# Autodesk Inventor assembly: CARCASA_ESTRUCTURA_Y_CHAPAS
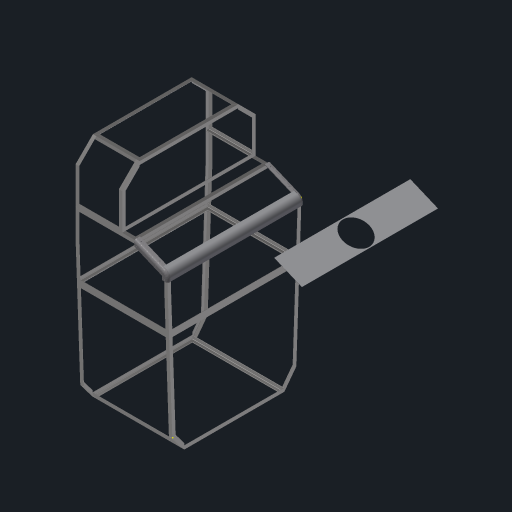
[picture p0: Inventor's stored thumbnail of the model, 512x512]
Saved by Autodesk Inventor 2024.3 (Build 283343000, 343)
## iProperties
Created: 2024-05-18
Part Number: CARCASA_ESTRUCTURA_Y_CHAPAS
Material: Generic
Document SubType Name: Assembly
Designer: Niler
Author: Niler
## Documents named in this file (11)
- C:\Users\Niler\OneDrive\Escritorio\RECICLADOR\RECICLADOR_MODELO_3D\VERSION_3_COMPLETA\CARCASA_ESTRUCTURA_Y_CHAPAS.iam
- C:\Users\Niler\OneDrive\Escritorio\RECICLADOR\RECICLADOR_MODELO_3D\VERSION_3_COMPLETA\ESTRUCTURA\ESTRUCTURA_COMPLETA.iam
- C:\Users\Niler\OneDrive\Escritorio\RECICLADOR\RECICLADOR_MODELO_3D\VERSION_3_COMPLETA\PIEZAS_CHAPAS_ALUMINIO\CARCASA_ALUM_2.ipt
- C:\Users\Niler\OneDrive\Escritorio\RECICLADOR\RECICLADOR_MODELO_3D\VERSION_3_COMPLETA\ESQUINAS\ESQUINA_REDONDEADA_R20_P1.ipt
- C:\Users\Niler\OneDrive\Escritorio\RECICLADOR\RECICLADOR_MODELO_3D\VERSION_3_COMPLETA\ESQUINAS\ESQUINA_REDONDEADA_R20_P2.ipt
- C:\Users\Niler\OneDrive\Escritorio\RECICLADOR\RECICLADOR_MODELO_3D\VERSION_3_COMPLETA\ESQUINAS\ESQUINA_REDONDEADA_R20_P3.ipt
- C:\Users\Niler\OneDrive\Escritorio\RECICLADOR\RECICLADOR_MODELO_3D\ESQUINA_REDONDEADA_R50.ipt
- C:\Users\Niler\OneDrive\Escritorio\RECICLADOR\RECICLADOR_MODELO_3D\ESQUINA_REDONDEADA_R50_P2.ipt
- C:\Users\Niler\OneDrive\Escritorio\RECICLADOR\RECICLADOR_MODELO_3D\VERSION_3_COMPLETA\ESQUINAS\ESQUINA_REDONDEADA_R20_P1_MIR.ipt
- C:\Users\Niler\OneDrive\Escritorio\RECICLADOR\RECICLADOR_MODELO_3D\VERSION_3_COMPLETA\ESQUINAS\ESQUINA_REDONDEADA_R20_P2_MIR.ipt
- C:\Users\Niler\OneDrive\Escritorio\RECICLADOR\RECICLADOR_MODELO_3D\VERSION_3_COMPLETA\ESQUINAS\ESQUINA_REDONDEADA_R20_P3_MIR.ipt
## Components (16 placed, 10 different names)
1. ESTRUCTURA_COMPLETA:1 [sub-assembly] — Mate:1, Mate:2, Angle:1, Mate:3, Angle:2, Mate:9, Mate:10, Mate:11, Mate:16, Mate:17, Mate:22, Mate:23, Mate:24, Mate:25
2. CARCASA_ALUM_2:1 — Mate:1
3. ESQUINA_REDONDEADA_R20_P1:1 — Mate:2, Angle:1, Mate:4, Mate:30
4. ESQUINA_REDONDEADA_R20_P2:1 — Mate:3, Angle:2, Mate:4, Mate:29
5. ESQUINA_REDONDEADA_R20_P3:1 — Mate:9, Mate:10, Mate:11, Flush:2, Flush:3, Flush:4, Mate:29, Mate:30
6. ESQUINA_REDONDEADA_R50:1 — Flush:2
7. ESQUINA_REDONDEADA_R50_P2:1 — Flush:3, Flush:4, Mate:27
8. ESQUINA_REDONDEADA_R20_P1_MIR:1 — Flush:5, Mate:13
9. ESQUINA_REDONDEADA_R20_P2_MIR:1 — Flush:5, Mate:13
10. ESQUINA_REDONDEADA_R20_P3_MIR:1
11. ESQUINA_REDONDEADA_R50:2 — Mate:14, Mate:15, Mate:16
12. ESQUINA_REDONDEADA_R50_P2:2 — Mate:14, Mate:15, Mate:17, Mate:27, Mate:28
13. ESQUINA_REDONDEADA_R50:3 — Mate:23, Mate:26
14. ESQUINA_REDONDEADA_R50_P2:3 — Mate:22, Mate:28
15. ESQUINA_REDONDEADA_R50:4 — Mate:24, Mate:26
16. ESQUINA_REDONDEADA_R50_P2:4 — Mate:25
## Relationships (31: Mate 25, Flush 4, Angle 2)
- Mate:1: ESTRUCTURA_COMPLETA:1 ↔ CARCASA_ALUM_2:1
- Mate:2: ESTRUCTURA_COMPLETA:1 ↔ ESQUINA_REDONDEADA_R20_P1:1
- Angle:1 (0 deg): ESTRUCTURA_COMPLETA:1 ↔ ESQUINA_REDONDEADA_R20_P1:1
- Mate:3: ESTRUCTURA_COMPLETA:1 ↔ ESQUINA_REDONDEADA_R20_P2:1
- Angle:2 (0 deg): ESTRUCTURA_COMPLETA:1 ↔ ESQUINA_REDONDEADA_R20_P2:1
- Mate:4: ESQUINA_REDONDEADA_R20_P1:1 ↔ ESQUINA_REDONDEADA_R20_P2:1
- Mate:9: ESTRUCTURA_COMPLETA:1 ↔ ESQUINA_REDONDEADA_R20_P3:1
- Mate:10: ESTRUCTURA_COMPLETA:1 ↔ ESQUINA_REDONDEADA_R20_P3:1
- Mate:11: ESTRUCTURA_COMPLETA:1 ↔ ESQUINA_REDONDEADA_R20_P3:1
- Flush:2: ESQUINA_REDONDEADA_R20_P3:1 ↔ ESQUINA_REDONDEADA_R50:1
- Flush:3: ESQUINA_REDONDEADA_R20_P3:1 ↔ ESQUINA_REDONDEADA_R50_P2:1
- Flush:4: ESQUINA_REDONDEADA_R20_P3:1 ↔ ESQUINA_REDONDEADA_R50_P2:1
- Flush:5: ESQUINA_REDONDEADA_R20_P1_MIR:1 ↔ ESQUINA_REDONDEADA_R20_P2_MIR:1
- Mate:13: ESQUINA_REDONDEADA_R20_P1_MIR:1 ↔ ESQUINA_REDONDEADA_R20_P2_MIR:1
- Mate:14: ESQUINA_REDONDEADA_R50:2 ↔ ESQUINA_REDONDEADA_R50_P2:2
- Mate:15: ESQUINA_REDONDEADA_R50:2 ↔ ESQUINA_REDONDEADA_R50_P2:2
- Mate:16: ESTRUCTURA_COMPLETA:1 ↔ ESQUINA_REDONDEADA_R50:2
- Mate:17: ESTRUCTURA_COMPLETA:1 ↔ ESQUINA_REDONDEADA_R50_P2:2
- [Mate]: ESQUINA_REDONDEADA_R50:3 ↔ ESQUINA_REDONDEADA_R50_P2:3
- [Mate]: ESQUINA_REDONDEADA_R50:3 ↔ ESQUINA_REDONDEADA_R50_P2:3
- [Mate]: ESQUINA_REDONDEADA_R50:4 ↔ ESQUINA_REDONDEADA_R50_P2:4
- [Mate]: ESQUINA_REDONDEADA_R50:4 ↔ ESQUINA_REDONDEADA_R50_P2:4
- Mate:22: ESTRUCTURA_COMPLETA:1 ↔ ESQUINA_REDONDEADA_R50_P2:3
- Mate:23: ESTRUCTURA_COMPLETA:1 ↔ ESQUINA_REDONDEADA_R50:3
- Mate:24: ESTRUCTURA_COMPLETA:1 ↔ ESQUINA_REDONDEADA_R50:4
- Mate:25: ESTRUCTURA_COMPLETA:1 ↔ ESQUINA_REDONDEADA_R50_P2:4
- Mate:26: ESQUINA_REDONDEADA_R50:3 ↔ ESQUINA_REDONDEADA_R50:4
- Mate:27: ESQUINA_REDONDEADA_R50_P2:1 ↔ ESQUINA_REDONDEADA_R50_P2:2
- Mate:28: ESQUINA_REDONDEADA_R50_P2:2 ↔ ESQUINA_REDONDEADA_R50_P2:3
- Mate:29: ESQUINA_REDONDEADA_R20_P2:1 ↔ ESQUINA_REDONDEADA_R20_P3:1
- Mate:30: ESQUINA_REDONDEADA_R20_P1:1 ↔ ESQUINA_REDONDEADA_R20_P3:1
## Named parameters: d31_d27 = 0 mm, d32_d28 = 0 mm, d33_d27 = 0 mm, d34_d28 = 0 mm
